# Autodesk Inventor assembly: scan_volume_M.cam_origin
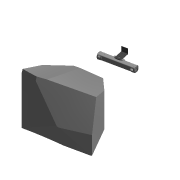
[picture p0: Inventor's stored thumbnail of the model, 180x180]
Saved by Autodesk Inventor 2019 (Build 230136000, 136)
## iProperties
Created: 2018-07-31
Part Number: scan_volume_M.cam_origin
Document SubType Name: Assembly
Designer: romanp
Sending System: Autodesk Translation Framework v7.1.0.215
Preprocessor: ST-DEVELOPER v17
Title: D:/scanners/Poslat_na_wiki_180731/scan_volume_M.step
Author: juranekUA8MM
## Documents named in this file (4)
- C:\Users\romanp\Downloads\actual_github_3d\3D\photoneo\scan_volume_M.cam_origin.iam
- C:\Users\romanp\Downloads\actual_github_3d\3D\photoneo\scan_volume_M_visible_space.ipt
- C:\Users\romanp\Downloads\actual_github_3d\3D\photoneo\assembly_M_2 v1.iam
- C:\Users\romanp\Downloads\actual_github_3d\3D\photoneo\Part5.ipt
## Components (3 placed, 3 different names)
1. scan_volume_M_visible_space:1
2. assembly_M_2 v1:1 [sub-assembly] — Insert:1, Insert:2
3. Part5:1 — Insert:1, Insert:2
## Relationships (2: Insert 2)
- Insert:1: assembly_M_2 v1:1 ↔ Part5:1
- Insert:2: assembly_M_2 v1:1 ↔ Part5:1
